# Autodesk Inventor assembly: Korpus
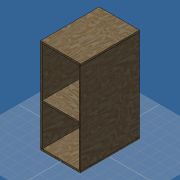
[picture p0: Inventor's stored thumbnail of the model, 180x180]
Saved by Autodesk Inventor 2019 (Build 230136000, 136)
## iProperties
Created: 2020-08-02
Part Number: Korpus
Material: Generisch
Document SubType Name: Assembly
Designer: Stefan
Mass: 36374.3 g
Surface Area: 43096.5 cm^2
Volume: 36374.3 cm^3
Density: 1 g/cm^3
Author: Stefan
## Documents named in this file (5)
- C:\Users\User\OneDrive\Dokumente\Inventor\Absauganlage\Korpus.iam
- C:\Users\User\OneDrive\Dokumente\Inventor\Absauganlage\Korpus_Basis.ipt
- C:\Users\User\OneDrive\Dokumente\Inventor\Absauganlage\Korpus_Seite.ipt
- C:\Users\User\OneDrive\Dokumente\Inventor\Absauganlage\Korpus_Rücken.ipt
- C:\Users\User\OneDrive\Dokumente\Inventor\Absauganlage\Korpus_Deckel.ipt
## Components (6 placed, 4 different names)
1. Korpus_Basis:1 — Passend:1, Fluchtend:1, Passend:3, Fluchtend:2, Passend:4, Passend:8
2. Korpus_Seite:1 — Passend:1, Fluchtend:1, Fluchtend:3, Passend:5, Fluchtend:4, Fluchtend:6, Passend:7, Fluchtend:8
3. Korpus_Seite:2 — Passend:3, Fluchtend:2, Fluchtend:3
4. Korpus_Rücken:1 — Passend:4, Passend:5, Fluchtend:4, Passend:6, Fluchtend:5, Fluchtend:7
5. Korpus_Deckel:1 — Passend:6, Fluchtend:5, Fluchtend:6
6. Korpus_Deckel:2 — Fluchtend:7, Passend:7, Fluchtend:8, Passend:8
## Relationships (15: Flush 8, Mate 7)
- Passend:1 [Mate]: Korpus_Basis:1 ↔ Korpus_Seite:1
- Fluchtend:1 [Flush]: Korpus_Basis:1 ↔ Korpus_Seite:1
- Passend:3 [Mate]: Korpus_Basis:1 ↔ Korpus_Seite:2
- Fluchtend:2 [Flush]: Korpus_Basis:1 ↔ Korpus_Seite:2
- Fluchtend:3 [Flush]: Korpus_Seite:1 ↔ Korpus_Seite:2
- Passend:4 [Mate]: Korpus_Basis:1 ↔ Korpus_Rücken:1
- Passend:5 [Mate]: Korpus_Seite:1 ↔ Korpus_Rücken:1
- Fluchtend:4 [Flush]: Korpus_Seite:1 ↔ Korpus_Rücken:1
- Passend:6 [Mate]: Korpus_Rücken:1 ↔ Korpus_Deckel:1
- Fluchtend:5 [Flush]: Korpus_Rücken:1 ↔ Korpus_Deckel:1
- Fluchtend:6 [Flush]: Korpus_Seite:1 ↔ Korpus_Deckel:1
- Fluchtend:7 [Flush]: Korpus_Rücken:1 ↔ Korpus_Deckel:2
- Passend:7 [Mate]: Korpus_Seite:1 ↔ Korpus_Deckel:2
- Fluchtend:8 [Flush]: Korpus_Seite:1 ↔ Korpus_Deckel:2
- Passend:8 [Mate] (400 mm): Korpus_Basis:1 ↔ Korpus_Deckel:2
